# Autodesk Inventor assembly: bottle capping machine
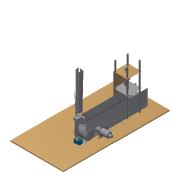
[picture p0: Inventor's stored thumbnail of the model, 180x180]
Saved by Autodesk Inventor 2019 (Build 230136000, 136)
## iProperties
Created: 2019-11-03
Part Number: bottle capping machine
Document SubType Name: Assembly
Designer: User
Author: User
## Documents named in this file (20)
- C:\Users\User\Documents\bottle capping machine.iam
- C:\Users\User\Documents\base.ipt
- C:\Users\User\Documents\conveyer belt.ipt
- C:\Users\User\Documents\roller.ipt
- C:\Users\User\Documents\sidesupport.ipt
- C:\Users\User\Documents\convermid.ipt
- C:\Users\User\Documents\capstoragees.ipt
- C:\Users\User\Documents\holder.ipt
- C:\Users\User\Documents\piston.ipt
- C:\Users\User\Documents\wood.ipt
- C:\Users\User\Documents\rods.ipt
- C:\Users\User\Documents\plate.ipt
- C:\Users\User\Documents\servos.ipt
- C:\Users\User\Documents\fixture.ipt
- C:\Users\User\Documents\servohandle.ipt
- C:\Users\User\Documents\dcmotor.ipt
- C:\Users\User\Documents\chuck.ipt
- C:\Users\User\Documents\secondside.ipt
- C:\Users\User\Documents\stand.ipt
- C:\Users\User\Documents\lclamp.ipt
## Components (31 placed, 19 different names)
1. base:1 — Mate:1, Mate:2, Mate:21, Mate:27, Mate:29, Mate:30, Mate:39
2. base:2 — Mate:1, Mate:2, Mate:4, Mate:6, Mate:11, Mate:13, Mate:15, Mate:17, Mate:19, Mate:32, Mate:35, Mate:37
3. conveyer belt:1
4. roller:1 — Mate:3, Mate:5
5. roller:2
6. convermid:1
7. sidesupport:4 — Mate:3, Mate:4, Mate:36, Mate:38
8. sidesupport:5 — Mate:5, Mate:6, Mate:31, Mate:33
9. capstoragees:1 — Mate:7, Mate:8, Mate:9
10. holder:2 — Mate:9
11. piston:4 — Mate:7, Mate:8, Mate:22
12. wood:1 — Mate:11, Mate:12, Mate:14, Mate:16, Mate:18, Mate:25, Mate:34
13. rods:1 — Mate:12, Mate:13
14. rods:2 — Mate:14, Mate:15, Mate:20
15. rods:3 — Mate:16, Mate:17
16. rods:4 — Mate:18, Mate:19
17. plate:1 — Mate:20, Mate:26
18. servos:1 — Mate:21, Mate:24
19. fixture:1 — Mate:22, Mate:23
20. servohandle:1 — Mate:23, Mate:24
21. dcmotor:1 — Mate:25
22. chuck:1 — Mate:26
23. secondside:1 — Mate:27, Mate:28
24. dcmotor:2 — Mate:28
25. holder:4
26. stand:1 — Mate:29
27. lclamp:1 — Mate:30, Mate:31
28. lclamp:2 — Mate:34, Mate:35
29. lclamp:3 — Mate:32, Mate:33
30. lclamp:5 — Mate:36, Mate:37
31. lclamp:6 — Mate:38, Mate:39
## Relationships (38: Mate 38)
- Mate:1: base:1 ↔ base:2
- Mate:2: base:1 ↔ base:2
- Mate:3: roller:1 ↔ sidesupport:4
- Mate:4: base:2 ↔ sidesupport:4
- Mate:5: roller:1 ↔ sidesupport:5
- Mate:6: base:2 ↔ sidesupport:5
- Mate:7: capstoragees:1 ↔ piston:4
- Mate:8: capstoragees:1 ↔ piston:4
- Mate:9: capstoragees:1 ↔ holder:2
- Mate:11: base:2 ↔ wood:1
- Mate:12: wood:1 ↔ rods:1
- Mate:13: base:2 ↔ rods:1
- Mate:14: wood:1 ↔ rods:2
- Mate:15: base:2 ↔ rods:2
- Mate:16: wood:1 ↔ rods:3
- Mate:17: base:2 ↔ rods:3
- Mate:18: wood:1 ↔ rods:4
- Mate:19: base:2 ↔ rods:4
- Mate:20: rods:2 ↔ plate:1
- Mate:21: base:1 ↔ servos:1
- Mate:22: piston:4 ↔ fixture:1
- Mate:23: fixture:1 ↔ servohandle:1
- Mate:24: servos:1 ↔ servohandle:1
- Mate:25: wood:1 ↔ dcmotor:1
- Mate:26: plate:1 ↔ chuck:1
- Mate:27: base:1 ↔ secondside:1
- Mate:28: secondside:1 ↔ dcmotor:2
- Mate:29: base:1 ↔ stand:1
- Mate:30: base:1 ↔ lclamp:1
- Mate:31: sidesupport:5 ↔ lclamp:1
- Mate:32: base:2 ↔ lclamp:3
- Mate:33: sidesupport:5 ↔ lclamp:3
- Mate:34: wood:1 ↔ lclamp:2
- Mate:35: base:2 ↔ lclamp:2
- Mate:36: sidesupport:4 ↔ lclamp:5
- Mate:37: base:2 ↔ lclamp:5
- Mate:38: sidesupport:4 ↔ lclamp:6
- Mate:39: base:1 ↔ lclamp:6
